# Autodesk Inventor assembly: Assembly4
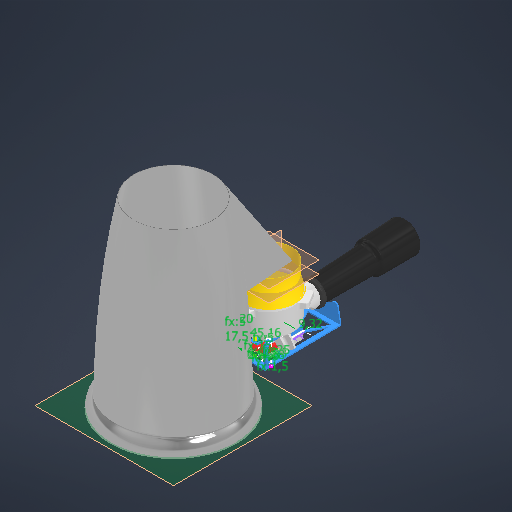
[picture p0: Inventor's stored thumbnail of the model, 512x512]
Saved by Autodesk Inventor 2026 (Build 300175000, 175)
## iProperties
Created: 2025-04-29
Part Number: Assembly4
Document SubType Name: Assembly
Designer: Paul Juschitz
Author: Paul Juschitz
## Documents named in this file (7)
- C:\Users\Paul Juschitz\Documents\private\m5_GBW_mod\M5_GBW_mod\CAD\Assembly4.iam
- C:\Users\Paul Juschitz\Documents\private\m5_GBW_mod\M5_GBW_mod\CAD\m2m_shell.ipt
- C:\Users\Paul Juschitz\Documents\private\m5_GBW_mod\M5_GBW_mod\CAD\load_cell_bracket.ipt
- C:\Users\Paul Juschitz\Documents\private\m5_GBW_mod\M5_GBW_mod\CAD\load_cell.ipt
- C:\Users\Paul Juschitz\Documents\private\m5_GBW_mod\M5_GBW_mod\CAD\my_portafilter_holder_7.ipt
- C:\Users\Paul Juschitz\Documents\private\m5_GBW_mod\M5_GBW_mod\CAD\downloads\portafilter\BES870XL Portafilter\BES870XL Portafilter\BES870XL Portafilter_assembled.iam
- C:\Users\Paul Juschitz\Documents\private\m5_GBW_mod\M5_GBW_mod\CAD\mock_dosing_funnel.ipt
## Components (6 placed, 6 different names)
1. m2m_shell:1 — Mate:1, Tangent:1, Flush:1
2. load_cell_bracket:1 — Mate:1, Tangent:1, Mate:2, Mate:3, Mate:4
3. load_cell:1 — Mate:2, Mate:3, Mate:4, Mate:5, Mate:6
4. my_portafilter_holder_7:1 — Mate:5, Mate:6, Tangent:2
5. BES870XL Portafilter_assembled:1 [sub-assembly] — Flush:1, Tangent:2, Mate:7
6. mock_dosing_funnel:1 — Mate:7
## Relationships (10: Mate 7, Tangent 2, Flush 1)
- Mate:1: m2m_shell:1 ↔ load_cell_bracket:1
- Tangent:1: m2m_shell:1 ↔ load_cell_bracket:1
- Mate:2: load_cell_bracket:1 ↔ load_cell:1
- Mate:3: load_cell_bracket:1 ↔ load_cell:1
- Mate:4: load_cell_bracket:1 ↔ load_cell:1
- Mate:5: load_cell:1 ↔ my_portafilter_holder_7:1
- Mate:6: load_cell:1 ↔ my_portafilter_holder_7:1
- Flush:1: m2m_shell:1 ↔ BES870XL Portafilter_assembled:1
- Tangent:2: my_portafilter_holder_7:1 ↔ BES870XL Portafilter_assembled:1
- Mate:7: BES870XL Portafilter_assembled:1 ↔ mock_dosing_funnel:1
